# Autodesk Inventor assembly: Trigger_Cell
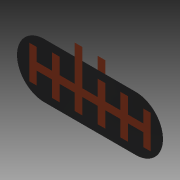
[picture p0: Inventor's stored thumbnail of the model, 180x180]
Saved by Autodesk Inventor 2014 SP1 (Build 180222100, 222)
## iProperties
Created: 2014-01-12
Part Number: Trigger_Cell
Document SubType Name: Assembly
Designer: tuleu
Author: tuleu
## Documents named in this file (3)
- C:\Users\tuleu\Documents\giant-snes-gamepad\cad\Trigger_Cell.iam
- C:\Users\tuleu\Documents\giant-snes-gamepad\cad\Trigger_Velostat.ipt
- C:\Users\tuleu\Documents\giant-snes-gamepad\cad\Trigger_Copper.ipt
## Components (3 placed, 2 different names)
1. Trigger_Velostat:1 — Mate:1, Flush:1, Mate:2, Mate:3, Mate:4, Mate:5
2. Trigger_Copper:1 — Mate:1, Flush:1, Mate:2
3. Trigger_Copper:2 — Mate:3, Mate:4, Mate:5
## Relationships (6: Mate 5, Flush 1)
- Mate:1: Trigger_Velostat:1 ↔ Trigger_Copper:1
- Flush:1: Trigger_Velostat:1 ↔ Trigger_Copper:1
- Mate:2: Trigger_Velostat:1 ↔ Trigger_Copper:1
- Mate:3: Trigger_Velostat:1 ↔ Trigger_Copper:2
- Mate:4: Trigger_Velostat:1 ↔ Trigger_Copper:2
- Mate:5: Trigger_Velostat:1 ↔ Trigger_Copper:2
